# Autodesk Inventor assembly: MIRleftMIRright脚四半
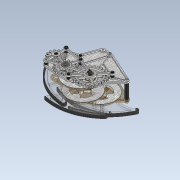
[picture p0: Inventor's stored thumbnail of the model, 180x180]
Saved by Autodesk Inventor 2020.2 (Build 242310000, 310)
## iProperties
Created: 2020-03-11
Part Number: MIRleftMIRright脚四半
Document SubType Name: Assembly
Designer: aoyama
Mass: 222.1 g
Surface Area: 1658.23 cm^2
Volume: 108.049 cm^3
Density: 2.05555 g/cm^3
Author: aoyam
## Documents named in this file (39)
- C:\Users\aoyam\Desktop\SRDC_local\Inventor\二年機\Geminiβ\脚\MIR達\MIRleftMIRright脚四半.iam
- C:\Users\aoyam\Desktop\SRDC_local\Inventor\二年機\Geminiβ\汎用部品\MIR達\MIRleftMIRrightワッシャD8d6m0.5.ipt
- C:\Users\aoyam\Desktop\SRDC_local\Inventor\二年機\Geminiβ\汎用部品\MIR達\MIRleftMIRrightワッシャD7d4m0.5.ipt
- C:\Users\aoyam\Desktop\SRDC_local\Inventor\二年機\Geminiβ\汎用部品\MIR達\MIRleftMIRrightｍ2歯数17ギアd3.99.ipt
- C:\Users\aoyam\Desktop\SRDC_local\Inventor\二年機\Geminiβ\汎用部品\MIR達\MIRleftMIRrightスペーサーM3L30アルミ.ipt
- C:\Users\aoyam\Desktop\SRDC_local\Inventor\二年機\Geminiβ\汎用部品\MIR達\MIRleftMIRrightネジボタンM3L6.ipt
- C:\Users\aoyam\Desktop\SRDC_local\Inventor\二年機\Geminiβ\汎用部品\MIR達\MIRleftMIRrightネジボタンM3L8.ipt
- C:\Users\aoyam\Desktop\SRDC_local\Inventor\二年機\Geminiβ\汎用部品\MIR達\MIRleftMIRrightスペーサーM3L30樹脂.ipt
- C:\Users\aoyam\Desktop\SRDC_local\Inventor\二年機\Geminiβ\汎用部品\MIR達\MIRleftMIRrightネジアルミM3L6.ipt
- C:\Users\aoyam\Desktop\SRDC_local\Inventor\二年機\Geminiβ\脚\ネジクランク\MIR達\MIRleftMIRright脚一枚1.iam
- C:\Users\aoyam\Desktop\SRDC_local\Inventor\二年機\Geminiβ\脚\ネジクランク\MIR達\MIRleftMIRrightカムL4F1.ipt
- C:\Users\aoyam\Desktop\SRDC_local\Inventor\二年機\Geminiβ\汎用部品\MIR達\MIRleftMIRrightオイレスドライメットFd10D12L3.ipt
- C:\Users\aoyam\Desktop\SRDC_local\Inventor\二年機\Geminiβ\汎用部品\MIR達\MIRleftMIRrightｍ2歯数25ギアネジ.ipt
- C:\Users\aoyam\Desktop\SRDC_local\Inventor\二年機\Geminiβ\脚\ネジクランク\MIR達\MIRleftMIRrightカムL31.ipt
- C:\Users\aoyam\Desktop\SRDC_local\Inventor\二年機\Geminiβ\汎用部品\MIR達\MIRleftMIRrightオイレスドライメットFd10D12L4.ipt
- C:\Users\aoyam\Desktop\SRDC_local\Inventor\二年機\Geminiβ\脚\ネジクランク\MIR達\MIRleftMIRrightカムL41.ipt
- C:\Users\aoyam\Desktop\SRDC_local\Inventor\二年機\Geminiβ\汎用部品\MIR達\MIRleftMIRrightネジキャップM3L45.ipt
- C:\Users\aoyam\Desktop\SRDC_local\Inventor\二年機\Geminiβ\汎用部品\MIR達\MIRleftMIRrightナットナイロンM3.ipt
- C:\Users\aoyam\Desktop\SRDC_local\Inventor\二年機\Geminiβ\汎用部品\MIR達\MIRleftMIRrightスペーサーM3L40アルミ.ipt
- C:\Users\aoyam\Desktop\SRDC_local\Inventor\二年機\Geminiβ\脚\MIR達\MIRleft脚フレーム外側前.ipt
- C:\Users\aoyam\Desktop\SRDC_local\Inventor\二年機\Geminiβ\汎用部品\MIR達\MIRleftオイレスFd6D8L7.ipt
- C:\Users\aoyam\Desktop\SRDC_local\Inventor\二年機\Geminiβ\汎用部品\MIR達\MIRleftネジ超極低頭M3L6.ipt
- C:\Users\aoyam\Desktop\SRDC_local\Inventor\二年機\Geminiβ\脚\脚フレーム内側前改.ipt
- C:\Users\aoyam\Desktop\SRDC_local\Inventor\二年機\Geminiβ\汎用部品\ｍ2歯数14ギアd12.ipt
- C:\Users\aoyam\Desktop\SRDC_local\Inventor\二年機\Geminiβ\汎用部品\ベアリングFd4D11B4.ipt
- C:\Users\aoyam\Desktop\SRDC_local\Inventor\二年機\Geminiβ\汎用部品\ワッシャD7d4m0.5.ipt
- C:\Users\aoyam\Desktop\SRDC_local\Inventor\二年機\Geminiβ\汎用部品\オイレスFd6D8L4.ipt
- C:\Users\aoyam\Desktop\SRDC_local\Inventor\二年機\Geminiβ\汎用部品\ベアリングFd6D12B4.ipt
- C:\Users\aoyam\Desktop\SRDC_local\Inventor\二年機\Geminiβ\汎用部品\ワッシャD10d6m0.3.ipt
- C:\Users\aoyam\Desktop\SRDC_local\Inventor\二年機\Geminiβ\汎用部品\ワッシャD8d6m0.5.ipt
- C:\Users\aoyam\Desktop\SRDC_local\Inventor\二年機\Geminiβ\汎用部品\オイレス外径8内径6L3.ipt
- C:\Users\aoyam\Desktop\SRDC_local\Inventor\二年機\Geminiβ\汎用部品\スペーサー中空M3L5樹脂.ipt
- C:\Users\aoyam\Desktop\SRDC_local\Inventor\二年機\Geminiβ\汎用部品\スペーサー中空M3L4樹脂.ipt
- C:\Users\aoyam\Desktop\SRDC_local\Inventor\二年機\Geminiβ\脚\脚ギアトレイン2.ipt
- C:\Users\aoyam\Desktop\SRDC_local\Inventor\二年機\Geminiβ\汎用部品\ネジ皿M3L8.ipt
- C:\Users\aoyam\Desktop\SRDC_local\Inventor\二年機\Geminiβ\汎用部品\ネジボタンM3L10.ipt
- C:\Users\aoyam\Desktop\SRDC_local\Inventor\二年機\Geminiβ\汎用部品\平行ピンD4L12.ipt
- C:\Users\aoyam\Desktop\SRDC_local\Inventor\二年機\Geminiβ\汎用部品\ネジキャップM3L15.ipt
- C:\Users\aoyam\Desktop\SRDC_local\Inventor\二年機\Geminiβ\汎用部品\ポリスラd6D14t0.25.ipt
## Components (61 placed, 38 different names)
1. MIRleftMIRrightワッシャD7d4m0.5:1 — 挿入:9, 挿入:86
2. MIRleftMIRrightｍ2歯数17ギアd3.99:1 — 挿入:9, 挿入:85
3. MIRleftMIRrightスペーサーM3L30アルミ:1 — 挿入:93, 挿入:88, メイト:13, メイト:12, メイト:11, メイト:10, 挿入:84
4. MIRleftMIRrightネジボタンM3L6:1 — 挿入:79
5. MIRleftMIRrightネジボタンM3L8:1 — 挿入:85
6. MIRleftMIRrightスペーサーM3L30樹脂:1 — 挿入:72, 挿入:82
7. MIRleftMIRrightスペーサーM3L30樹脂:2 — 挿入:71, 挿入:81
8. MIRleftMIRrightワッシャD8d6m0.5:3 — 挿入:93, 挿入:129
9. MIRleftMIRrightワッシャD8d6m0.5:4 — 挿入:88, 挿入:130
10. MIRleftMIRrightワッシャD8d6m0.5:5 — 挿入:129
11. MIRleftMIRrightネジアルミM3L6:1 — 挿入:76
12. MIRleftMIRrightネジアルミM3L6:2 — 挿入:77
13. MIRleftMIRrightネジアルミM3L6:3 — 挿入:86
14. MIRleftMIRrightネジアルミM3L6:4 — 挿入:87
15. MIRleftMIRright脚一枚1:1 [sub-assembly] — メイト:13, 挿入:103, 挿入:104, 挿入:109, 挿入:110, 挿入:94
16. MIRleftMIRright脚一枚1:2 [sub-assembly] — メイト:12, 挿入:103, 挿入:104, 挿入:105, 挿入:106, 挿入:93
17. MIRleftMIRright脚一枚1:3 [sub-assembly] — メイト:11, 挿入:105, 挿入:106, 挿入:107, 挿入:108, 挿入:92
18. MIRleftMIRright脚一枚1:4 [sub-assembly] — メイト:10, 挿入:107, 挿入:108, メイト:6, メイト:7, 挿入:91
19. MIRleftMIRrightカムL4F1:1 — 挿入:109, 挿入:110, 挿入:112, 挿入:119, 挿入:120
20. MIRleftMIRrightオイレスドライメットFd10D12L3:1 — 挿入:112, 挿入:89
21. MIRleftMIRrightｍ2歯数25ギアネジ:1 — メイト:6, 挿入:114, 挿入:115, 挿入:116, 挿入:99
22. MIRleftMIRrightオイレスドライメットFd10D12L3:2 — 挿入:114
23. MIRleftMIRrightカムL31:1 — 挿入:115, 挿入:116, 挿入:121, 挿入:122
24. MIRleftMIRrightオイレスドライメットFd10D12L4:1 — 挿入:118, 挿入:80, 挿入:99
25. MIRleftMIRrightカムL41:1 — 挿入:118, メイト:7
26. MIRleftMIRrightネジキャップM3L45:1 — 挿入:119
27. MIRleftMIRrightネジキャップM3L45:2 — 挿入:120
28. MIRleftMIRrightナットナイロンM3:1 — 挿入:121, メイト:8
29. MIRleftMIRrightナットナイロンM3:2 — 挿入:122, メイト:8
30. MIRleftMIRrightスペーサーM3L40アルミ:1 — 挿入:96, 挿入:94
31. MIRleftMIRrightワッシャD8d6m0.5:6 — 挿入:130
32. MIRleft脚フレーム外側前:1 — 挿入:89, 挿入:87, 挿入:86, 挿入:85, 挿入:84, 挿入:81, 挿入:82
33. MIRleftオイレスFd6D8L7:1 — 挿入:91
34. MIRleftオイレスFd6D8L7:2 — 挿入:92
35. MIRleftオイレスFd6D8L7:3 — 挿入:93
36. MIRleftオイレスFd6D8L7:4 — 挿入:94
37. MIRleftネジ超極低頭M3L6:1 — 挿入:96
38. 脚フレーム内側前改:1 — 挿入:71, 挿入:72, 挿入:76, 挿入:77, 挿入:79, 挿入:80, 挿入:83, 挿入:87, 挿入:95, 挿入:96, 挿入:97, 挿入:98, 挿入:104
39. ｍ2歯数14ギアd12:1 — 挿入:90
40. ベアリングFd4D11B4:1 — 挿入:83, 挿入:84
41. ベアリングFd4D11B4:2 — 挿入:86, 挿入:109
42. ワッシャD7d4m0.5:1 — 挿入:84, 挿入:85
43. オイレスFd6D8L4:1 — 挿入:87, 挿入:91
44. ベアリングFd6D12B4:1 — 挿入:90, 挿入:92
45. ワッシャD10d6m0.3:1 — 挿入:92, 挿入:93
46. ワッシャD8d6m0.5:1 — 挿入:91
47. オイレス外径8内径6L3:1 — 挿入:93, 挿入:112
48. スペーサー中空M3L5樹脂:1 — 挿入:95
49. スペーサー中空M3L5樹脂:2 — 挿入:97, 挿入:102
50. スペーサー中空M3L5樹脂:3 — 挿入:96, 挿入:101
51. スペーサー中空M3L5樹脂:4 — 挿入:98, 挿入:100
52. スペーサー中空M3L4樹脂:1 — 挿入:94, 挿入:103
53. 脚ギアトレイン2:1 — 挿入:100, 挿入:101, 挿入:102, 挿入:103, 挿入:105, 挿入:107, 挿入:108, 挿入:110
54. ネジ皿M3L8:1 — 挿入:104
55. ネジボタンM3L10:1 — 挿入:105
56. ネジボタンM3L10:2 — 挿入:108
57. ネジボタンM3L10:3 — 挿入:107
58. 平行ピンD4L12:1 — 挿入:109
59. ネジキャップM3L15:1 — 挿入:110
60. ポリスラd6D14t0.25:1 — 挿入:111, 挿入:112
61. ポリスラd6D14t0.25:2 — 挿入:111
## Relationships (74: Insert 67, Mate 7)
- 挿入:9 [Insert]: MIRleftMIRrightワッシャD7d4m0.5:1 ↔ MIRleftMIRrightｍ2歯数17ギアd3.99:1
- 挿入:93 [Insert]: MIRleftMIRrightスペーサーM3L30アルミ:1 ↔ MIRleftMIRrightワッシャD8d6m0.5:3
- 挿入:88 [Insert]: MIRleftMIRrightスペーサーM3L30アルミ:1 ↔ MIRleftMIRrightワッシャD8d6m0.5:4
- 挿入:129 [Insert]: MIRleftMIRrightワッシャD8d6m0.5:3 ↔ MIRleftMIRrightワッシャD8d6m0.5:5
- メイト:13 [Mate]: MIRleftMIRrightスペーサーM3L30アルミ:1 ↔ MIRleftMIRright脚一枚1:1
- メイト:12 [Mate]: MIRleftMIRrightスペーサーM3L30アルミ:1 ↔ MIRleftMIRright脚一枚1:2
- 挿入:103 [Insert]: MIRleftMIRright脚一枚1:1 ↔ MIRleftMIRright脚一枚1:2
- 挿入:104 [Insert]: MIRleftMIRright脚一枚1:1 ↔ MIRleftMIRright脚一枚1:2
- メイト:11 [Mate]: MIRleftMIRrightスペーサーM3L30アルミ:1 ↔ MIRleftMIRright脚一枚1:3
- 挿入:105 [Insert]: MIRleftMIRright脚一枚1:2 ↔ MIRleftMIRright脚一枚1:3
- 挿入:106 [Insert]: MIRleftMIRright脚一枚1:2 ↔ MIRleftMIRright脚一枚1:3
- メイト:10 [Mate]: MIRleftMIRrightスペーサーM3L30アルミ:1 ↔ MIRleftMIRright脚一枚1:4
- 挿入:107 [Insert]: MIRleftMIRright脚一枚1:3 ↔ MIRleftMIRright脚一枚1:4
- 挿入:108 [Insert]: MIRleftMIRright脚一枚1:3 ↔ MIRleftMIRright脚一枚1:4
- 挿入:109 [Insert]: MIRleftMIRright脚一枚1:1 ↔ MIRleftMIRrightカムL4F1:1
- 挿入:110 [Insert]: MIRleftMIRright脚一枚1:1 ↔ MIRleftMIRrightカムL4F1:1
- 挿入:112 [Insert]: MIRleftMIRrightカムL4F1:1 ↔ MIRleftMIRrightオイレスドライメットFd10D12L3:1
- メイト:6 [Mate]: MIRleftMIRright脚一枚1:4 ↔ MIRleftMIRrightｍ2歯数25ギアネジ:1
- 挿入:114 [Insert]: MIRleftMIRrightｍ2歯数25ギアネジ:1 ↔ MIRleftMIRrightオイレスドライメットFd10D12L3:2
- 挿入:115 [Insert]: MIRleftMIRrightｍ2歯数25ギアネジ:1 ↔ MIRleftMIRrightカムL31:1
- 挿入:116 [Insert]: MIRleftMIRrightｍ2歯数25ギアネジ:1 ↔ MIRleftMIRrightカムL31:1
- 挿入:118 [Insert]: MIRleftMIRrightオイレスドライメットFd10D12L4:1 ↔ MIRleftMIRrightカムL41:1
- メイト:7 [Mate]: MIRleftMIRright脚一枚1:4 ↔ MIRleftMIRrightカムL41:1
- 挿入:119 [Insert]: MIRleftMIRrightカムL4F1:1 ↔ MIRleftMIRrightネジキャップM3L45:1
- 挿入:120 [Insert]: MIRleftMIRrightカムL4F1:1 ↔ MIRleftMIRrightネジキャップM3L45:2
- 挿入:121 [Insert]: MIRleftMIRrightカムL31:1 ↔ MIRleftMIRrightナットナイロンM3:1
- 挿入:122 [Insert]: MIRleftMIRrightカムL31:1 ↔ MIRleftMIRrightナットナイロンM3:2
- メイト:8 [Mate]: MIRleftMIRrightナットナイロンM3:1 ↔ MIRleftMIRrightナットナイロンM3:2
- 挿入:130 [Insert]: MIRleftMIRrightワッシャD8d6m0.5:4 ↔ MIRleftMIRrightワッシャD8d6m0.5:6
- 挿入:89 [Insert]: MIRleftMIRrightオイレスドライメットFd10D12L3:1 ↔ MIRleft脚フレーム外側前:1
- 挿入:87 [Insert]: MIRleftMIRrightネジアルミM3L6:4 ↔ MIRleft脚フレーム外側前:1
- 挿入:86 [Insert]: MIRleftMIRrightネジアルミM3L6:3 ↔ MIRleft脚フレーム外側前:1
- 挿入:85 [Insert]: MIRleftMIRrightネジボタンM3L8:1 ↔ MIRleft脚フレーム外側前:1
- 挿入:84 [Insert]: MIRleftMIRrightスペーサーM3L30アルミ:1 ↔ MIRleft脚フレーム外側前:1
- 挿入:91 [Insert]: MIRleftMIRright脚一枚1:4 ↔ MIRleftオイレスFd6D8L7:1
- 挿入:92 [Insert]: MIRleftMIRright脚一枚1:3 ↔ MIRleftオイレスFd6D8L7:2
- 挿入:93 [Insert]: MIRleftMIRright脚一枚1:2 ↔ MIRleftオイレスFd6D8L7:3
- 挿入:94 [Insert]: MIRleftMIRright脚一枚1:1 ↔ MIRleftオイレスFd6D8L7:4
- 挿入:96 [Insert]: MIRleftMIRrightスペーサーM3L40アルミ:1 ↔ MIRleftネジ超極低頭M3L6:1
- 挿入:71 [Insert]: MIRleftMIRrightスペーサーM3L30樹脂:2 ↔ 脚フレーム内側前改:1
- 挿入:72 [Insert]: MIRleftMIRrightスペーサーM3L30樹脂:1 ↔ 脚フレーム内側前改:1
- 挿入:76 [Insert]: MIRleftMIRrightネジアルミM3L6:1 ↔ 脚フレーム内側前改:1
- 挿入:77 [Insert]: MIRleftMIRrightネジアルミM3L6:2 ↔ 脚フレーム内側前改:1
- 挿入:79 [Insert]: MIRleftMIRrightネジボタンM3L6:1 ↔ 脚フレーム内側前改:1
- 挿入:80 [Insert]: MIRleftMIRrightオイレスドライメットFd10D12L4:1 ↔ 脚フレーム内側前改:1
- 挿入:81 [Insert]: MIRleftMIRrightスペーサーM3L30樹脂:2 ↔ MIRleft脚フレーム外側前:1
- 挿入:82 [Insert]: MIRleftMIRrightスペーサーM3L30樹脂:1 ↔ MIRleft脚フレーム外側前:1
- 挿入:83 [Insert]: 脚フレーム内側前改:1 ↔ ベアリングFd4D11B4:1
- 挿入:84 [Insert]: ベアリングFd4D11B4:1 ↔ ワッシャD7d4m0.5:1
- 挿入:85 [Insert]: MIRleftMIRrightｍ2歯数17ギアd3.99:1 ↔ ワッシャD7d4m0.5:1
- 挿入:86 [Insert]: MIRleftMIRrightワッシャD7d4m0.5:1 ↔ ベアリングFd4D11B4:2
- 挿入:87 [Insert]: 脚フレーム内側前改:1 ↔ オイレスFd6D8L4:1
- 挿入:90 [Insert]: ｍ2歯数14ギアd12:1 ↔ ベアリングFd6D12B4:1
- 挿入:91 [Insert]: オイレスFd6D8L4:1 ↔ ワッシャD8d6m0.5:1
- 挿入:92 [Insert]: ベアリングFd6D12B4:1 ↔ ワッシャD10d6m0.3:1
- 挿入:93 [Insert]: ワッシャD10d6m0.3:1 ↔ オイレス外径8内径6L3:1
- 挿入:94 [Insert]: MIRleftMIRrightスペーサーM3L40アルミ:1 ↔ スペーサー中空M3L4樹脂:1
- 挿入:95 [Insert]: 脚フレーム内側前改:1 ↔ スペーサー中空M3L5樹脂:1
- 挿入:96 [Insert]: 脚フレーム内側前改:1 ↔ スペーサー中空M3L5樹脂:3
- 挿入:97 [Insert]: 脚フレーム内側前改:1 ↔ スペーサー中空M3L5樹脂:2
- 挿入:98 [Insert]: 脚フレーム内側前改:1 ↔ スペーサー中空M3L5樹脂:4
- 挿入:99 [Insert]: MIRleftMIRrightｍ2歯数25ギアネジ:1 ↔ MIRleftMIRrightオイレスドライメットFd10D12L4:1
- 挿入:100 [Insert]: スペーサー中空M3L5樹脂:4 ↔ 脚ギアトレイン2:1
- 挿入:101 [Insert]: スペーサー中空M3L5樹脂:3 ↔ 脚ギアトレイン2:1
- 挿入:102 [Insert]: スペーサー中空M3L5樹脂:2 ↔ 脚ギアトレイン2:1
- 挿入:103 [Insert]: スペーサー中空M3L4樹脂:1 ↔ 脚ギアトレイン2:1
- 挿入:104 [Insert]: 脚フレーム内側前改:1 ↔ ネジ皿M3L8:1
- 挿入:105 [Insert]: 脚ギアトレイン2:1 ↔ ネジボタンM3L10:1
- 挿入:107 [Insert]: 脚ギアトレイン2:1 ↔ ネジボタンM3L10:3
- 挿入:108 [Insert]: 脚ギアトレイン2:1 ↔ ネジボタンM3L10:2
- 挿入:109 [Insert]: ベアリングFd4D11B4:2 ↔ 平行ピンD4L12:1
- 挿入:110 [Insert]: 脚ギアトレイン2:1 ↔ ネジキャップM3L15:1
- 挿入:111 [Insert]: ポリスラd6D14t0.25:1 ↔ ポリスラd6D14t0.25:2
- 挿入:112 [Insert]: オイレス外径8内径6L3:1 ↔ ポリスラd6D14t0.25:1
